# Autodesk Inventor assembly: Attempt2
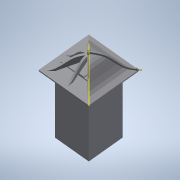
[picture p0: Inventor's stored thumbnail of the model, 180x180]
Saved by Autodesk Inventor 2020.2 (Build 242310000, 310)
## iProperties
Created: 2020-12-28
Part Number: Attempt2
Document SubType Name: Assembly
Designer: Thomas Dodd
Author: Thomas Dodd
## Documents named in this file (18)
- C:\Users\Thomas J H Dodd\OneDrive - Millfield Enterprises Limited\Millfield\2020\Joachim's Salmon Smoker\Joachim's Roof\Attempt2 - Copy.iam
- C:\Users\Thomas J H Dodd\OneDrive - Millfield Enterprises Limited\Millfield\2020\Joachim's Salmon Smoker\Joachim's Roof\Box.ipt
- C:\Users\Thomas J H Dodd\OneDrive - Millfield Enterprises Limited\Millfield\2020\Joachim's Salmon Smoker\Joachim's Roof\Lower Base Plate.ipt
- C:\Users\Thomas J H Dodd\OneDrive - Millfield Enterprises Limited\Millfield\2020\Joachim's Salmon Smoker\Joachim's Roof\Upper Base Plate.ipt
- C:\Users\Thomas J H Dodd\OneDrive - Millfield Enterprises Limited\Millfield\2020\Joachim's Salmon Smoker\Joachim's Roof\Main Beam.ipt
- C:\Users\Thomas J H Dodd\OneDrive - Millfield Enterprises Limited\Millfield\2020\Joachim's Salmon Smoker\Joachim's Roof\Secondary Beam.ipt
- C:\Users\Thomas J H Dodd\OneDrive - Millfield Enterprises Limited\Millfield\2020\Joachim's Salmon Smoker\Joachim's Roof\Central Part.ipt
- C:\Users\Thomas J H Dodd\OneDrive - Millfield Enterprises Limited\Millfield\2020\Joachim's Salmon Smoker\Joachim's Roof\Panel1.ipt
- C:\Users\Thomas J H Dodd\OneDrive - Millfield Enterprises Limited\Millfield\2020\Joachim's Salmon Smoker\Joachim's Roof\Panel2.ipt
- C:\Users\Thomas J H Dodd\OneDrive - Millfield Enterprises Limited\Millfield\2020\Joachim's Salmon Smoker\Joachim's Roof\Panel3.ipt
- C:\Users\Thomas J H Dodd\OneDrive - Millfield Enterprises Limited\Millfield\2020\Joachim's Salmon Smoker\Joachim's Roof\Panel4.ipt
- C:\Users\Thomas J H Dodd\OneDrive - Millfield Enterprises Limited\Millfield\2020\Joachim's Salmon Smoker\Joachim's Roof\Panel5.ipt
- C:\Users\Thomas J H Dodd\OneDrive - Millfield Enterprises Limited\Millfield\2020\Joachim's Salmon Smoker\Joachim's Roof\Panel6.ipt
- C:\Users\Thomas J H Dodd\OneDrive - Millfield Enterprises Limited\Millfield\2020\Joachim's Salmon Smoker\Joachim's Roof\Panel7.ipt
- C:\Users\Thomas J H Dodd\OneDrive - Millfield Enterprises Limited\Millfield\2020\Joachim's Salmon Smoker\Joachim's Roof\Panel8.ipt
- C:\Users\Thomas J H Dodd\OneDrive - Millfield Enterprises Limited\Millfield\2020\Joachim's Salmon Smoker\Joachim's Roof\Cross Support 1.ipt
- C:\Users\Thomas J H Dodd\OneDrive - Millfield Enterprises Limited\Millfield\2020\Joachim's Salmon Smoker\Joachim's Roof\Cross Support 2.ipt
- C:\Users\Thomas J H Dodd\OneDrive - Millfield Enterprises Limited\Millfield\2020\Joachim's Salmon Smoker\Joachim's Roof\Cover Beam Final.ipt
## Components (38 placed, 17 different names)
1. Box:1 — Mate:1, Mate:2, Flush:3
2. Lower Base Plate:1 — Rigid:2
3. Lower Base Plate:2 — Rigid:2, Rigid:3, Mate:3
4. Lower Base Plate:3 — Rigid:1, Mate:2, Flush:2
5. Lower Base Plate:4 — Rigid:1, Rigid:3, Mate:1, Flush:1
6. Upper Base Plate:1 — Rigid:5, Rigid:6, Mate:3, Mate:9, Mate:12, Flush:9
7. Upper Base Plate:2 — Rigid:5, Flush:3, Mate:7, Mate:8, Flush:8, Mate:11, Rigid:7, Flush:16
8. Upper Base Plate:3 — Rigid:4, Flush:2, Mate:10, Flush:10, Rigid:8, Flush:17
9. Upper Base Plate:4 — Rigid:4, Rigid:6, Flush:1, Mate:6, Mate:13, Mate:27, Mate:29, Flush:12
10. Main Beam:1 — Flush:4, Flush:5, Mate:15, Mate:24, Mate:25
11. Main Beam:2 — Flush:4, Flush:5, Mate:7, Mate:8, Mate:17, Mate:19, Mate:22
12. Main Beam:3 — Flush:6, Flush:7, Mate:16, Mate:20, Mate:26
13. Main Beam:4 — Flush:6, Flush:7, Mate:6, Mate:9, Mate:14, Mate:21, Mate:23
14. Secondary Beam:1 — Mate:11, Mate:19, Mate:20
15. Secondary Beam:2 — Mate:10, Mate:25, Mate:26
16. Secondary Beam:3 — Mate:12, Mate:21, Mate:22
17. Secondary Beam:4 — Mate:13, Mate:23, Mate:24, Mate:28, Mate:30
18. Central Part:1 — Mate:14, Mate:15, Mate:16, Mate:17, Flush:9, Flush:10, Mate:34
19. Panel1:3 — Rigid:7, Rigid:10
20. Panel1:4 — Rigid:8, Rigid:9, Mate:33
21. Panel2:2 — Rigid:10, Rigid:12
22. Panel2:3 — Rigid:9, Rigid:11
23. Panel3:1 — Rigid:12, Rigid:14
24. Panel3:2 — Rigid:11, Rigid:13
25. Panel4:1 — Rigid:13, Rigid:16
26. Panel4:2 — Rigid:14, Rigid:15
27. Panel5:1 — Rigid:15, Rigid:18
28. Panel5:2 — Rigid:16, Rigid:17
29. Panel6:1 — Rigid:17, Rigid:19
30. Panel6:2 — Rigid:18, Rigid:20
31. Panel7:1 — Rigid:19, Rigid:21
32. Panel7:2 — Rigid:20, Rigid:22
33. Panel8:1 — Rigid:22, Flush:15
34. Panel8:2 — Rigid:21
35. Cross Support 1:1 — Mate:27, Mate:28, Flush:11, Flush:12, Mate:31, Flush:14
36. Cross Support 1:2 — Mate:29, Mate:30, Flush:11, Flush:13
37. Cross Support 2:1 — Mate:31, Flush:13, Flush:14, Mate:34
38. Cover Beam Final:1 — Flush:16, Flush:17, Mate:33
## Relationships (69: Mate 30, WeldJoint 22, Flush 17)
- Rigid:1 [WeldJoint]: Lower Base Plate:3 ↔ Lower Base Plate:4
- Rigid:2 [WeldJoint]: Lower Base Plate:1 ↔ Lower Base Plate:2
- Rigid:3 [WeldJoint]: Lower Base Plate:2 ↔ Lower Base Plate:4
- Mate:1: Box:1 ↔ Lower Base Plate:4
- Mate:2: Box:1 ↔ Lower Base Plate:3
- Rigid:4 [WeldJoint]: Upper Base Plate:3 ↔ Upper Base Plate:4
- Rigid:5 [WeldJoint]: Upper Base Plate:1 ↔ Upper Base Plate:2
- Rigid:6 [WeldJoint]: Upper Base Plate:1 ↔ Upper Base Plate:4
- Mate:3: Lower Base Plate:2 ↔ Upper Base Plate:1
- Flush:1: Lower Base Plate:4 ↔ Upper Base Plate:4
- Flush:2: Lower Base Plate:3 ↔ Upper Base Plate:3
- Flush:3: Box:1 ↔ Upper Base Plate:2
- Flush:4: Main Beam:1 ↔ Main Beam:2
- Flush:5: Main Beam:1 ↔ Main Beam:2
- Flush:6: Main Beam:3 ↔ Main Beam:4
- Flush:7: Main Beam:3 ↔ Main Beam:4
- Mate:6 (-20 mm): Upper Base Plate:4 ↔ Main Beam:4
- Mate:7 (-20 mm): Upper Base Plate:2 ↔ Main Beam:2
- Mate:8: Upper Base Plate:2 ↔ Main Beam:2
- Mate:9: Upper Base Plate:1 ↔ Main Beam:4
- Flush:8 (-445 mm): Upper Base Plate:2
- Mate:10: Upper Base Plate:3 ↔ Secondary Beam:2
- Mate:11: Upper Base Plate:2 ↔ Secondary Beam:1
- Mate:12: Upper Base Plate:1 ↔ Secondary Beam:3
- Mate:13: Upper Base Plate:4 ↔ Secondary Beam:4
- Mate:14: Main Beam:4 ↔ Central Part:1
- Mate:15: Main Beam:1 ↔ Central Part:1
- Mate:16: Main Beam:3 ↔ Central Part:1
- Mate:17: Main Beam:2 ↔ Central Part:1
- Flush:9 (-20 mm): Upper Base Plate:1 ↔ Central Part:1
- Flush:10 (-20 mm): Upper Base Plate:3 ↔ Central Part:1
- Mate:19: Main Beam:2 ↔ Secondary Beam:1
- Mate:20: Main Beam:3 ↔ Secondary Beam:1
- Mate:21: Main Beam:4 ↔ Secondary Beam:3
- Mate:22: Main Beam:2 ↔ Secondary Beam:3
- Mate:23: Main Beam:4 ↔ Secondary Beam:4
- Mate:24: Main Beam:1 ↔ Secondary Beam:4
- Mate:25: Main Beam:1 ↔ Secondary Beam:2
- Mate:26: Main Beam:3 ↔ Secondary Beam:2
- Rigid:7 [WeldJoint]: Upper Base Plate:2 ↔ Panel1:3
- Rigid:8 [WeldJoint]: Upper Base Plate:3 ↔ Panel1:4
- Rigid:9 [WeldJoint]: Panel1:4 ↔ Panel2:3
- Rigid:10 [WeldJoint]: Panel1:3 ↔ Panel2:2
- Rigid:11 [WeldJoint]: Panel2:3 ↔ Panel3:2
- Rigid:12 [WeldJoint]: Panel2:2 ↔ Panel3:1
- Rigid:13 [WeldJoint]: Panel3:2 ↔ Panel4:1
- Rigid:14 [WeldJoint]: Panel3:1 ↔ Panel4:2
- Rigid:15 [WeldJoint]: Panel4:2 ↔ Panel5:1
- Rigid:16 [WeldJoint]: Panel4:1 ↔ Panel5:2
- Rigid:17 [WeldJoint]: Panel5:2 ↔ Panel6:1
- Rigid:18 [WeldJoint]: Panel5:1 ↔ Panel6:2
- Rigid:19 [WeldJoint]: Panel6:1 ↔ Panel7:1
- Rigid:20 [WeldJoint]: Panel6:2 ↔ Panel7:2
- Rigid:21 [WeldJoint]: Panel7:1 ↔ Panel8:2
- Rigid:22 [WeldJoint]: Panel7:2 ↔ Panel8:1
- Mate:27: Upper Base Plate:4 ↔ Cross Support 1:1
- Mate:28: Secondary Beam:4 ↔ Cross Support 1:1
- Mate:29: Upper Base Plate:4 ↔ Cross Support 1:2
- Mate:30: Secondary Beam:4 ↔ Cross Support 1:2
- Flush:11: Cross Support 1:1 ↔ Cross Support 1:2
- Flush:12 (105 mm): Upper Base Plate:4 ↔ Cross Support 1:1
- Mate:31: Cross Support 1:1 ↔ Cross Support 2:1
- Flush:13 (270 mm): Cross Support 1:2 ↔ Cross Support 2:1
- Flush:14: Cross Support 1:1 ↔ Cross Support 2:1
- Flush:15: Panel8:1
- Flush:16: Upper Base Plate:2 ↔ Cover Beam Final:1
- Flush:17: Upper Base Plate:3 ↔ Cover Beam Final:1
- Mate:33: Panel1:4 ↔ Cover Beam Final:1
- Mate:34: Central Part:1 ↔ Cross Support 2:1
